# Autodesk Inventor assembly: omniwheel_complete
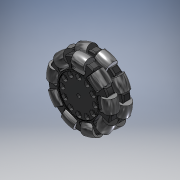
[picture p0: Inventor's stored thumbnail of the model, 180x180]
Saved by Autodesk Inventor 2018 (Build 220112000, 112)
## iProperties
Created: 2011-12-02
Part Number: omniwheel_complete
Document SubType Name: Assembly
Designer: AYUSH SHUKLA
Sending System: SolidWorks 2014
Last Author: SKP
Last Saved: 2015-06-20
Author: AYUSH SHUKLA
## Documents named in this file (3)
- C:\Study\BTP2\Robomuse Inventor CAD\castor\omniwheel_complete.iam
- C:\Study\BTP2\Robomuse Inventor CAD\castor\omniwheel_1.ipt
- C:\Study\BTP2\Robomuse Inventor CAD\castor\subwheel.ipt
## Components (20 placed, 2 different names)
1. omniwheel_1:1 — Mate:1, Mate:2, Mate:3, Mate:4, Mate:5, Mate:8, Mate:9, Mate:10, Mate:11, Mate:12, Mate:13, Mate:14, Mate:15, Mate:16, Mate:17, Mate:18, Mate:19, Mate:20, Mate:21, Mate:22, Mate:23
2. omniwheel_1:3 — Mate:3, Mate:4, Mate:5, Mate:6, Mate:7, Mate:24, Mate:25, Mate:26, Mate:27, Mate:28, Mate:29, Mate:30, Mate:31, Mate:32, Mate:33, Mate:34, Mate:35, Mate:36, Mate:37, Mate:38, Mate:39
3. subwheel:1 — Mate:8, Mate:9
4. subwheel:2 — Mate:22, Mate:23
5. subwheel:3 — Mate:1, Mate:2
6. subwheel:4 — Mate:20, Mate:21
7. subwheel:5 — Mate:18, Mate:19
8. subwheel:6 — Mate:16, Mate:17
9. subwheel:7 — Mate:14, Mate:15
10. subwheel:8 — Mate:12, Mate:13
11. subwheel:9 — Mate:10, Mate:11
12. subwheel:10 — Mate:28, Mate:29
13. subwheel:11 — Mate:30, Mate:31
14. subwheel:12 — Mate:6, Mate:7
15. subwheel:13 — Mate:32, Mate:33
16. subwheel:14 — Mate:34, Mate:35
17. subwheel:15 — Mate:36, Mate:37
18. subwheel:16 — Mate:38, Mate:39
19. subwheel:17 — Mate:24, Mate:25
20. subwheel:18 — Mate:26, Mate:27
## Relationships (39: Mate 39)
- Mate:1: omniwheel_1:1 ↔ subwheel:3
- Mate:2 (1 mm): omniwheel_1:1 ↔ subwheel:3
- Mate:3: omniwheel_1:1 ↔ omniwheel_1:3
- Mate:4: omniwheel_1:1 ↔ omniwheel_1:3
- Mate:5 (9 mm): omniwheel_1:1 ↔ omniwheel_1:3
- Mate:6: omniwheel_1:3 ↔ subwheel:12
- Mate:7 (1 mm): omniwheel_1:3 ↔ subwheel:12
- Mate:8: omniwheel_1:1 ↔ subwheel:1
- Mate:9 (1 mm): omniwheel_1:1 ↔ subwheel:1
- Mate:10: omniwheel_1:1 ↔ subwheel:9
- Mate:11 (1 mm): omniwheel_1:1 ↔ subwheel:9
- Mate:12: omniwheel_1:1 ↔ subwheel:8
- Mate:13 (1 mm): omniwheel_1:1 ↔ subwheel:8
- Mate:14: omniwheel_1:1 ↔ subwheel:7
- Mate:15 (1 mm): omniwheel_1:1 ↔ subwheel:7
- Mate:16: omniwheel_1:1 ↔ subwheel:6
- Mate:17 (1 mm): omniwheel_1:1 ↔ subwheel:6
- Mate:18: omniwheel_1:1 ↔ subwheel:5
- Mate:19 (1 mm): omniwheel_1:1 ↔ subwheel:5
- Mate:20: omniwheel_1:1 ↔ subwheel:4
- Mate:21 (1 mm): omniwheel_1:1 ↔ subwheel:4
- Mate:22: omniwheel_1:1 ↔ subwheel:2
- Mate:23 (1 mm): omniwheel_1:1 ↔ subwheel:2
- Mate:24: omniwheel_1:3 ↔ subwheel:17
- Mate:25 (1 mm): omniwheel_1:3 ↔ subwheel:17
- Mate:26: omniwheel_1:3 ↔ subwheel:18
- Mate:27 (1 mm): omniwheel_1:3 ↔ subwheel:18
- Mate:28: omniwheel_1:3 ↔ subwheel:10
- Mate:29 (1 mm): omniwheel_1:3 ↔ subwheel:10
- Mate:30: omniwheel_1:3 ↔ subwheel:11
- Mate:31 (1 mm): omniwheel_1:3 ↔ subwheel:11
- Mate:32: omniwheel_1:3 ↔ subwheel:13
- Mate:33 (1 mm): omniwheel_1:3 ↔ subwheel:13
- Mate:34: omniwheel_1:3 ↔ subwheel:14
- Mate:35 (1 mm): omniwheel_1:3 ↔ subwheel:14
- Mate:36: omniwheel_1:3 ↔ subwheel:15
- Mate:37 (1 mm): omniwheel_1:3 ↔ subwheel:15
- Mate:38: omniwheel_1:3 ↔ subwheel:16
- Mate:39 (1 mm): omniwheel_1:3 ↔ subwheel:16
